# Autodesk Inventor assembly: Shooter assembly
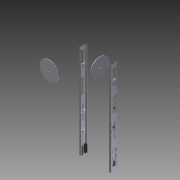
[picture p0: Inventor's stored thumbnail of the model, 180x180]
Saved by Autodesk Inventor 2014 SP1 (Build 180222100, 222)
## iProperties
Created: 2014-02-21
Part Number: Shooter assembly
Document SubType Name: Assembly
Designer: Asif
Author: Asif
## Documents named in this file (6)
- C:\Users\Asif\Documents\GitHub\CAD\CAD Team 2014\Shooter\Shooter assembly.iam
- C:\Users\Asif\Documents\GitHub\CAD\CAD Team 2014\Shooter\U-CHANNEL 6 Sot_sheet metal Edited to size.ipt
- C:\Users\Asif\Documents\GitHub\CAD\CAD Team 2014\Shooter\8020-1010 edited to size.ipt
- C:\Users\Asif\Documents\GitHub\CAD\CAD Team 2014\Shooter\CIM RECEIVER - AM-0860.ipt
- C:\Users\Asif\Documents\GitHub\CAD\CAD Team 2014\Shooter\3-8 bearing.ipt
- C:\Users\Asif\Documents\GitHub\CAD\CAD Team 2014\Shooter\80t Sprocket.ipt
## Components (20 placed, 5 different names)
1. U-CHANNEL 6 Sot_sheet metal Edited to size:1 — Mate:1, Mate:2, Mate:3, Mate:4, Flush:2, Flush:5, Flush:6, Flush:7, Mate:9, Mate:16, Mate:17, Mate:18, Mate:19, Mate:20
2. U-CHANNEL 6 Sot_sheet metal Edited to size:2 — Mate:5, Mate:6, Flush:3, Mate:7, Mate:8, Flush:4, Flush:6, Flush:7, Mate:10, Mate:11, Mate:12, Mate:13, Mate:14, Mate:15
3. 8020-1010 edited to size:1 — Mate:3, Mate:4, Flush:2
4. 8020-1010 edited to size:2 — Mate:1, Mate:2, Flush:5, Tangent:1
5. 8020-1010 edited to size:3 — Mate:5, Mate:6, Flush:3, Tangent:1
6. 8020-1010 edited to size:4 — Mate:7, Mate:8, Flush:4
7. CIM RECEIVER - AM-0860:1 — Mate:9, Mate:18, Insert:8
8. CIM RECEIVER - AM-0860:2 — Mate:14, Mate:15, Insert:4
9. CIM RECEIVER - AM-0860:3 — Mate:10, Mate:11, Insert:7
10. CIM RECEIVER - AM-0860:4 — Mate:12, Mate:13, Insert:6
11. CIM RECEIVER - AM-0860:5 — Mate:19, Mate:20, Insert:3
12. CIM RECEIVER - AM-0860:6 — Mate:16, Mate:17, Insert:1
13. 3-8 bearing:1 — Insert:6
14. 3-8 bearing:2 — Insert:4
15. 3-8 bearing:3 — Insert:7
16. 3-8 bearing:4 — Insert:1, Planar:1
17. 3-8 bearing:5 — Insert:3
18. 3-8 bearing:6 — Insert:8
19. 80t Sprocket:1 — Planar:1
20. 80t Sprocket:2
## Relationships (34: Mate 20, Flush 6, Insert 6, Tangent 1, PlanarJoint 1)
- Mate:1: U-CHANNEL 6 Sot_sheet metal Edited to size:1 ↔ 8020-1010 edited to size:2
- Mate:2: U-CHANNEL 6 Sot_sheet metal Edited to size:1 ↔ 8020-1010 edited to size:2
- Mate:3: U-CHANNEL 6 Sot_sheet metal Edited to size:1 ↔ 8020-1010 edited to size:1
- Mate:4: U-CHANNEL 6 Sot_sheet metal Edited to size:1 ↔ 8020-1010 edited to size:1
- Flush:2: U-CHANNEL 6 Sot_sheet metal Edited to size:1 ↔ 8020-1010 edited to size:1
- Mate:5: U-CHANNEL 6 Sot_sheet metal Edited to size:2 ↔ 8020-1010 edited to size:3
- Mate:6: U-CHANNEL 6 Sot_sheet metal Edited to size:2 ↔ 8020-1010 edited to size:3
- Flush:3: U-CHANNEL 6 Sot_sheet metal Edited to size:2 ↔ 8020-1010 edited to size:3
- Mate:7: U-CHANNEL 6 Sot_sheet metal Edited to size:2 ↔ 8020-1010 edited to size:4
- Mate:8: U-CHANNEL 6 Sot_sheet metal Edited to size:2 ↔ 8020-1010 edited to size:4
- Flush:4: U-CHANNEL 6 Sot_sheet metal Edited to size:2 ↔ 8020-1010 edited to size:4
- Flush:5: U-CHANNEL 6 Sot_sheet metal Edited to size:1 ↔ 8020-1010 edited to size:2
- Flush:6: U-CHANNEL 6 Sot_sheet metal Edited to size:1 ↔ U-CHANNEL 6 Sot_sheet metal Edited to size:2
- Flush:7: U-CHANNEL 6 Sot_sheet metal Edited to size:1 ↔ U-CHANNEL 6 Sot_sheet metal Edited to size:2
- Tangent:1 (381 mm): 8020-1010 edited to size:2 ↔ 8020-1010 edited to size:3
- Mate:9: U-CHANNEL 6 Sot_sheet metal Edited to size:1 ↔ CIM RECEIVER - AM-0860:1
- Mate:10: U-CHANNEL 6 Sot_sheet metal Edited to size:2 ↔ CIM RECEIVER - AM-0860:3
- Mate:11: U-CHANNEL 6 Sot_sheet metal Edited to size:2 ↔ CIM RECEIVER - AM-0860:3
- Mate:12: U-CHANNEL 6 Sot_sheet metal Edited to size:2 ↔ CIM RECEIVER - AM-0860:4
- Mate:13: U-CHANNEL 6 Sot_sheet metal Edited to size:2 ↔ CIM RECEIVER - AM-0860:4
- Mate:14: U-CHANNEL 6 Sot_sheet metal Edited to size:2 ↔ CIM RECEIVER - AM-0860:2
- Mate:15: U-CHANNEL 6 Sot_sheet metal Edited to size:2 ↔ CIM RECEIVER - AM-0860:2
- Mate:16: U-CHANNEL 6 Sot_sheet metal Edited to size:1 ↔ CIM RECEIVER - AM-0860:6
- Mate:17: U-CHANNEL 6 Sot_sheet metal Edited to size:1 ↔ CIM RECEIVER - AM-0860:6
- Mate:18: U-CHANNEL 6 Sot_sheet metal Edited to size:1 ↔ CIM RECEIVER - AM-0860:1
- Mate:19: U-CHANNEL 6 Sot_sheet metal Edited to size:1 ↔ CIM RECEIVER - AM-0860:5
- Mate:20: U-CHANNEL 6 Sot_sheet metal Edited to size:1 ↔ CIM RECEIVER - AM-0860:5
- Insert:1: CIM RECEIVER - AM-0860:6 ↔ 3-8 bearing:4
- Insert:3: CIM RECEIVER - AM-0860:5 ↔ 3-8 bearing:5
- Insert:4: CIM RECEIVER - AM-0860:2 ↔ 3-8 bearing:2
- Insert:6: CIM RECEIVER - AM-0860:4 ↔ 3-8 bearing:1
- Insert:7: CIM RECEIVER - AM-0860:3 ↔ 3-8 bearing:3
- Insert:8: CIM RECEIVER - AM-0860:1 ↔ 3-8 bearing:6
- Planar:1: 3-8 bearing:4 ↔ 80t Sprocket:1
